# Autodesk Inventor assembly: Wheels on Chassis Assembly
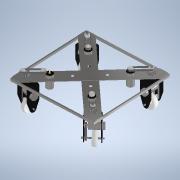
[picture p0: Inventor's stored thumbnail of the model, 180x180]
Saved by Autodesk Inventor 2020 (Build 240168000, 168)
## iProperties
Created: 2022-07-06
Part Number: Wheels on Chassis Assembly
Document SubType Name: Assembly
Designer: karimi2
Author: karimi2
## Documents named in this file (8)
- C:\Users\karimi2\Documents\PROJECT\src\Wheels on Chassis Assembly.iam
- C:\Users\karimi2\Documents\PROJECT\src\Chassis.ipt
- C:\Users\karimi2\Documents\PROJECT\src\Wheel Assembly.iam
- C:\Users\karimi2\Documents\PROJECT\src\GearedDCmotor.ipt
- C:\Users\karimi2\Documents\PROJECT\src\Assembly1\Design Accelerator\Synchronous Belts Transmission1.iam
- C:\Users\karimi2\Documents\PROJECT\src\Assembly1\Design Accelerator\Synchronous Belts Transmission2.iam
- C:\Users\karimi2\Documents\PROJECT\src\Assembly1\Design Accelerator\Synchronous Belts Transmission3.iam
- C:\Users\karimi2\Documents\PROJECT\src\Assembly1\Design Accelerator\Synchronous Belts Transmission4.iam
## Components (13 placed, 4 different names)
1. Chassis:1 — Mate:1, Rotational:1, Mate:2, Rigid:1, Mate:3, Rotational:2, Mate:4, Rotational:3, Mate:5, Rotational:4, Mate:6, Rigid:2, Mate:7, Rigid:3, Mate:8, Rigid:4
2. Wheel Assembly:1 [sub-assembly] — Mate:1, Rotational:1
3. GearedDCmotor:1 — Mate:2, Rigid:1
4. Synchronous Belts Transmission:1 [sub-assembly]
5. Wheel Assembly:2 [sub-assembly] — Mate:3, Rotational:2
6. Wheel Assembly:3 [sub-assembly] — Mate:4, Rotational:3
7. Wheel Assembly:4 [sub-assembly] — Mate:5, Rotational:4
8. GearedDCmotor:2 — Mate:6, Rigid:2
9. GearedDCmotor:3 — Mate:7, Rigid:3
10. GearedDCmotor:4 — Mate:8, Rigid:4
11. Synchronous Belts Transmission:2 [sub-assembly]
12. Synchronous Belts Transmission:3 [sub-assembly]
13. Synchronous Belts Transmission:4 [sub-assembly]
## Relationships (16: Mate 8, RevoluteJoint 4, WeldJoint 4)
- Mate:1: Chassis:1 ↔ Wheel Assembly:1
- Rotational:1 [RevoluteJoint] (-3.5 mm): Chassis:1 ↔ Wheel Assembly:1
- Mate:2: Chassis:1 ↔ GearedDCmotor:1
- Rigid:1 [WeldJoint] (-6 mm): Chassis:1 ↔ GearedDCmotor:1
- Mate:3: Chassis:1 ↔ Wheel Assembly:2
- Rotational:2 [RevoluteJoint] (-3.5 mm): Chassis:1 ↔ Wheel Assembly:2
- Mate:4: Chassis:1 ↔ Wheel Assembly:3
- Rotational:3 [RevoluteJoint] (-3.5 mm): Chassis:1 ↔ Wheel Assembly:3
- Mate:5: Chassis:1 ↔ Wheel Assembly:4
- Rotational:4 [RevoluteJoint] (-3.5 mm): Chassis:1 ↔ Wheel Assembly:4
- Mate:6: Chassis:1 ↔ GearedDCmotor:2
- Rigid:2 [WeldJoint] (-6 mm): Chassis:1 ↔ GearedDCmotor:2
- Mate:7: Chassis:1 ↔ GearedDCmotor:3
- Rigid:3 [WeldJoint] (-6 mm): Chassis:1 ↔ GearedDCmotor:3
- Mate:8: Chassis:1 ↔ GearedDCmotor:4
- Rigid:4 [WeldJoint] (-6 mm): Chassis:1 ↔ GearedDCmotor:4
